# Autodesk Inventor assembly: Механизм подъема
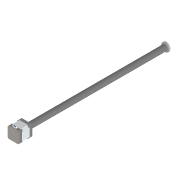
[picture p0: Inventor's stored thumbnail of the model, 180x180]
Saved by Autodesk Inventor 2022 (Build 260153000, 153)
## iProperties
Created: 2023-02-20
Part Number: Механизм подъема
Document SubType Name: Assembly
Designer: Глеб
Author: Глеб
## Documents named in this file (3)
- C:\Users\Глеб\Documents\Inventor\Файлы Inventor\Механизм подъема.iam
- C:\Users\Глеб\Documents\Inventor\Файлы Inventor\NEMA17_STEPPER.ipt
- C:\Users\Глеб\Documents\Inventor\Файлы Inventor\Резьбовой винт.ipt
## Components (2 placed, 2 different names)
1. NEMA17_STEPPER:1 — Совмещение:1, Совмещение:2
2. Резьбовой винт:1 — Совмещение:1, Совмещение:2
## Relationships (2: Mate 2)
- Совмещение:1 [Mate]: NEMA17_STEPPER:1 ↔ Резьбовой винт:1
- Совмещение:2 [Mate]: NEMA17_STEPPER:1 ↔ Резьбовой винт:1
